# Autodesk Inventor assembly: rev2
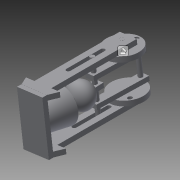
[picture p0: Inventor's stored thumbnail of the model, 180x180]
Saved by Autodesk Inventor 2015 (Build 190159000, 159)
## iProperties
Created: 2014-07-15
Part Number: rev2
Document SubType Name: Assembly
Designer: shohei
Author: shohei
## Documents named in this file (10)
- C:\Users\shohei\Documents\Inventor\FufuPounder\rev2.iam
- C:\Users\shohei\Documents\Inventor\FufuPounder\mortar.ipt
- C:\Users\shohei\Documents\Inventor\FufuPounder\Part1.ipt
- C:\Users\shohei\Documents\Inventor\FufuPounder\Part2.ipt
- C:\Users\shohei\Documents\Inventor\FufuPounder\pulley.ipt
- C:\Users\shohei\Documents\Inventor\FufuPounder\Part4.ipt
- C:\Users\shohei\Documents\Inventor\FufuPounder\baseboard.ipt
- C:\Users\shohei\Documents\Inventor\FufuPounder\shaft2.ipt
- C:\Users\shohei\Documents\Inventor\FufuPounder\shaft3.ipt
- C:\Users\shohei\Documents\Inventor\FufuPounder\mallet_aseembly.iam
## Components (13 placed, 9 different names)
1. mortar:1
2. Part1:1 — Flush:3, Mate:4, Flush:5, Slider:1, Rotational:9
3. Part1:2 — Flush:3, Mate:2, Mate:3, Flush:4, Mate:5, Rigid:1
4. pulley:1 — Cylindrical:12, Angle:1, Cylindrical:15, Cylindrical:17, Cylindrical:19
5. Part4:1 — Rotational:3, Cylindrical:16
6. Part4:2 — Rotational:7, Rotational:8
7. Part2:3 — Rigid:1, Cylindrical:17
8. baseboard:1 — Mate:2, Mate:3, Mate:4, Flush:4, Mate:5, Flush:5, Angle:1
9. shaft2:1 — Cylindrical:14, Rotational:3, Slider:1, Rotational:7
10. shaft3:1 — Cylindrical:12, Cylindrical:15, Rotational:8, Cylindrical:16, Cylindrical:19
11. mallet_aseembly:1 [sub-assembly] — Cylindrical:14
12. pulley:2 — Cylindrical:18
13. Part2:5 — Rotational:9, Cylindrical:18
## Relationships (21: CylindricalJoint 7, Mate 4, RevoluteJoint 4, Flush 3, Angle 1, TranslationJoint 1, WeldJoint 1)
- Flush:3: Part1:1 ↔ Part1:2
- Mate:2: Part1:2 ↔ baseboard:1
- Mate:3: Part1:2 ↔ baseboard:1
- Mate:4: Part1:1 ↔ baseboard:1
- Flush:4: Part1:2 ↔ baseboard:1
- Mate:5: Part1:2 ↔ baseboard:1
- Flush:5: Part1:1 ↔ baseboard:1
- Cylindrical:12: pulley:1 ↔ shaft3:1
- Cylindrical:14: shaft2:1 ↔ mallet_aseembly:1
- Angle:1 (2000 deg): pulley:1 ↔ baseboard:1
- Rotational:3 [RevoluteJoint] (-20 mm): Part4:1 ↔ shaft2:1
- Cylindrical:15: pulley:1 ↔ shaft3:1
- Slider:1 [TranslationJoint]: Part1:1 ↔ shaft2:1
- Rotational:7 [RevoluteJoint] (-12.5 mm): Part4:2 ↔ shaft2:1
- Rotational:8 [RevoluteJoint]: Part4:2 ↔ shaft3:1
- Cylindrical:16: Part4:1 ↔ shaft3:1
- Rigid:1 [WeldJoint]: Part1:2 ↔ Part2:3
- Cylindrical:17: pulley:1 ↔ Part2:3
- Rotational:9 [RevoluteJoint]: Part1:1 ↔ Part2:5
- Cylindrical:18: pulley:2 ↔ Part2:5
- Cylindrical:19: pulley:1 ↔ shaft3:1
